# Autodesk Inventor assembly: Assembly
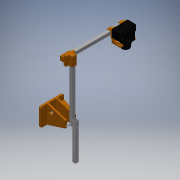
[picture p0: Inventor's stored thumbnail of the model, 180x180]
Saved by Autodesk Inventor 2019.3 (Build 233278000, 278)
## iProperties
Created: 2019-06-24
Part Number: Assembly
Document SubType Name: Assembly
Designer: mark
Author: mark
## Documents named in this file (10)
- D:\git\photometric-leds\Mechanical\Assembly.iam
- D:\git\photometric-leds\Mechanical\Canon_Rebel_T3i.ipt
- D:\git\photometric-leds\Mechanical\RailMount.ipt
- D:\git\photometric-leds\Mechanical\LateralBars.ipt
- D:\git\photometric-leds\Mechanical\CornerBracket.ipt
- D:\git\photometric-leds\Mechanical\RailMountSupport.ipt
- D:\git\photometric-leds\Mechanical\VerticalBar.ipt
- D:\git\photometric-leds\Mechanical\MotorSupport.ipt
- D:\git\photometric-leds\Mechanical\CameraBracket.ipt
- D:\git\photometric-leds\Mechanical\CounterWeight.ipt
## Components (10 placed, 9 different names)
1. Canon_Rebel_T3i:1 — Flush:1, Insert:1
2. CameraBracket:1 — Flush:1, Flush:2, Insert:1, Flush:5
3. RailMount:1 — Flush:2, Mate:1, Mate:2, Mate:3
4. LateralBars:1 — Mate:1, Mate:2, Mate:3, Mate:4, Mate:5, Mate:6
5. VerticalBar:1 — Mate:8, Mate:9, Mate:10, Flush:6, Flush:7
6. CornerBracket:1 — Mate:7, Flush:3, Flush:4, Mate:8, Mate:9, Mate:10
7. CornerBracket:2 — Mate:4, Mate:5, Mate:6, Mate:7, Flush:3, Flush:4
8. RailMountSupport:1 — Flush:5
9. MotorSupport:1 — Flush:6
10. CounterWeight:1 — Flush:7
## Relationships (18: Mate 10, Flush 7, Insert 1)
- Flush:1: Canon_Rebel_T3i:1 ↔ CameraBracket:1
- Flush:2: CameraBracket:1 ↔ RailMount:1
- Insert:1: Canon_Rebel_T3i:1 ↔ CameraBracket:1
- Mate:1: RailMount:1 ↔ LateralBars:1
- Mate:2: RailMount:1 ↔ LateralBars:1
- Mate:3: RailMount:1 ↔ LateralBars:1
- Mate:4: LateralBars:1 ↔ CornerBracket:2
- Mate:5: LateralBars:1 ↔ CornerBracket:2
- Mate:6: LateralBars:1 ↔ CornerBracket:2
- Mate:7: CornerBracket:1 ↔ CornerBracket:2
- Flush:3: CornerBracket:1 ↔ CornerBracket:2
- Flush:4: CornerBracket:1 ↔ CornerBracket:2
- Flush:5: CameraBracket:1 ↔ RailMountSupport:1
- Mate:8: VerticalBar:1 ↔ CornerBracket:1
- Mate:9: VerticalBar:1 ↔ CornerBracket:1
- Mate:10: VerticalBar:1 ↔ CornerBracket:1
- Flush:6 (17.3 mm): VerticalBar:1 ↔ MotorSupport:1
- Flush:7: VerticalBar:1 ↔ CounterWeight:1
